# Autodesk Inventor assembly: DragBarLinkage3 Full Assembly
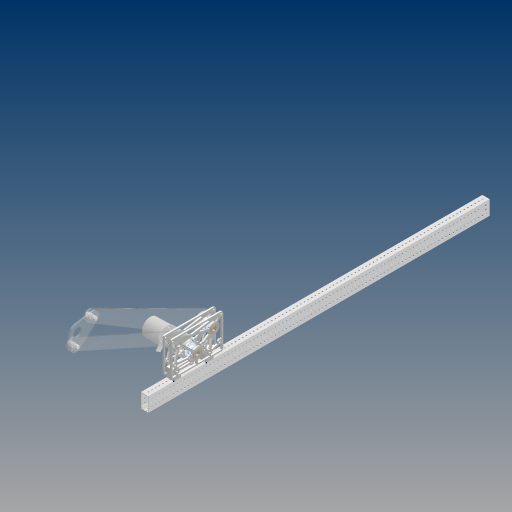
[picture p0: Inventor's stored thumbnail of the model, 512x512]
Saved by Autodesk Inventor 2024.3 (Build 283343000, 343)
## iProperties
Created: 2024-07-08
Part Number: DragBarLinkage3 Full Assembly
Document SubType Name: Assembly
Designer: Kenji
Author: Kenji
## Documents named in this file (21)
- C:\Users\Kenji\Documents\FRC\Offseason 2024\DragBarLinkage3\DragBarLinkage3 Full Assembly.iam
- C:\Users\Kenji\Documents\FRC\Offseason 2024\DragBarLinkage3\MAXPlanetary 3-Stage2.iam
- C:\Users\Kenji\Documents\FRC\Offseason 2024\DragBarLinkage3\DragBarLinkage3 Bar1.ipt
- C:\Users\Kenji\Documents\FRC\Offseason 2024\DragBarLinkage3\DragBarLinkage3 Bar2.ipt
- C:\Users\Kenji\Documents\FRC\Offseason 2024\DragBarLinkage3\DragBarLinkage3 Bar3.ipt
- C:\Users\Kenji\Documents\FRC\Offseason 2024\DragBarLinkage3\REV-21-2289.ipt
- C:\Users\Kenji\Documents\FRC\Offseason 2024\DragBarLinkage3\6655K14_Thrust Ball Bearing.ipt
- C:\Users\Kenji\Documents\FRC\Offseason 2024\DragBarLinkage3\57155K306_Stainless Steel Ball Bearing.ipt
- C:\Users\Kenji\Documents\FRC\Offseason 2024\DragBarLinkage3\91259A581_Alloy Steel Shoulder Screw.ipt
- C:\Users\Kenji\Documents\FRC\Offseason 2024\DragBarLinkage3\92141A226_18-8 Stainless Steel Washer.ipt
- C:\Users\Kenji\Documents\FRC\Offseason 2024\DragBarLinkage3\97135A414_High-Strength Steel Nylon-Insert Locknut.ipt
- C:\Users\Kenji\Documents\FRC\Offseason 2024\DragBarLinkage3\DragBarLinkage3 Bracket1.ipt
- C:\Users\Kenji\Documents\FRC\Offseason 2024\DragBarLinkage3\DragBarLinkage3 Billet.ipt
- C:\Users\Kenji\Documents\FRC\Offseason 2024\DragBarLinkage3\WCP-0754.ipt
- C:\Users\Kenji\Documents\FRC\Offseason 2024\DragBarLinkage3\WCP-0783 (1).ipt
- C:\Users\Kenji\Documents\FRC\Offseason 2024\DragBarLinkage3\1_2” Hex Bore Aluminum VersaHub (217-2592).ipt
- C:\Users\Kenji\Documents\FRC\Offseason 2024\DragBarLinkage3\5909K978_1-16 Thick Washe.ipt
- C:\Users\Kenji\Documents\FRC\Offseason 2024\DragBarLinkage3\5909K24_Needle-Roller Thrust Bearing.ipt
- C:\Users\Kenji\Documents\FRC\Offseason 2024\DragBarLinkage3\5909K951_Needle-Roller Thrust Bearing.ipt
- C:\Users\Kenji\Documents\FRC\Offseason 2024\DragBarLinkage3\5909K979_1-16 Thick Washe.ipt
- C:\Users\Kenji\Documents\FRC\Offseason 2024\DragBarLinkage3\5909K971_1-32 Thick Washe.ipt
## Components (36 placed, 20 different names)
1. MAXPlanetary 3-Stage2:1 [sub-assembly] — Mate:51, Mate:53, Mate:67
2. DragBarLinkage3 Bar1:1 — Mate:4, Mate:5, Mate:13, Mate:54, Mate:77, Mate:78, Mate:79
3. DragBarLinkage3 Bar2:1 — Mate:16, Mate:17, Mate:18, Mate:19, Mate:20, Mate:21, Mate:22, Mate:23
4. DragBarLinkage3 Bar3:1 — Mate:6, Mate:7, Mate:14, Mate:15, Mate:55, Mate:81, Mate:90, Mate:91, Mate:92
5. REV-21-2289:1 — Mate:41, Mate:42, Mate:43, Mate:44, Flush:1
6. 6655K14_Thrust Ball Bearing:1 — Mate:14, Mate:15, Mate:22, Mate:23
7. 6655K14_Thrust Ball Bearing:2 — Mate:12, Mate:13, Mate:20, Mate:21
8. 57155K306_Stainless Steel Ball Bearing:5 — Mate:16, Mate:18, Mate:36
9. 57155K306_Stainless Steel Ball Bearing:6 — Mate:6, Mate:7, Mate:26, Mate:27
10. 57155K306_Stainless Steel Ball Bearing:7 — Mate:4, Mate:5, Mate:12, Mate:24, Mate:25
11. 57155K306_Stainless Steel Ball Bearing:8 — Mate:17, Mate:19, Mate:31
12. 91259A581_Alloy Steel Shoulder Screw:1 — Mate:28, Mate:29, Mate:30
13. 91259A581_Alloy Steel Shoulder Screw:2 — Mate:32, Mate:33, Mate:34, Mate:35
14. 92141A226_18-8 Stainless Steel Washer:1 — Mate:24, Mate:25, Mate:28, Mate:29
15. 92141A226_18-8 Stainless Steel Washer:2 — Mate:26, Mate:27, Mate:32, Mate:33
16. 97135A414_High-Strength Steel Nylon-Insert Locknut:1 — Mate:30, Mate:31
17. 97135A414_High-Strength Steel Nylon-Insert Locknut:2 — Mate:34, Mate:35, Mate:36
18. DragBarLinkage3 Bracket1:2 — Mate:59, Mate:60, Mate:61, Mate:69, Mate:70, Mate:73, Mate:74
19. DragBarLinkage3 Billet:1 — Mate:42, Mate:44, Flush:2, Mate:50, Mate:58, Mate:60, Mate:61
20. DragBarLinkage3 Billet:2 — Mate:41, Mate:43, Flush:1, Flush:2, Mate:57, Mate:59
21. DragBarLinkage3 Bracket1:3 — Mate:50, Mate:51, Mate:53, Mate:54, Mate:55, Mate:57, Mate:58, Mate:66, Mate:67, Mate:68, Mate:71, Mate:72, Mate:76, Mate:80, Mate:82, Mate:83
22. 57155K306_Stainless Steel Ball Bearing:9 — Mate:81, Mate:82, Mate:88, Mate:89
23. 57155K306_Stainless Steel Ball Bearing:10 — Mate:80, Mate:83
24. WCP-0754:1 — Mate:66, Mate:76
25. WCP-0754:2 — Mate:68, Mate:75
26. WCP-0783 (1):1 — Mate:73, Mate:74
27. WCP-0783 (1):2 — Mate:71, Mate:72, Mate:75, Mate:98, Mate:99
28. WCP-0783 (1):4 — Mate:69, Mate:70
29. 1_2” Hex Bore Aluminum VersaHub (217-2592):1 — Mate:77, Mate:78, Mate:79
30. 5909K978_1-16 Thick Washe:1 — Mate:84, Mate:87, Mate:88, Mate:90
31. 5909K978_1-16 Thick Washe:2 — Mate:85, Mate:86, Mate:89
32. 5909K24_Needle-Roller Thrust Bearing:1 — Mate:84, Mate:85, Mate:86, Mate:87
33. 57155K306_Stainless Steel Ball Bearing:11 — Mate:91, Mate:92
34. 5909K951_Needle-Roller Thrust Bearing:1 — Mate:93, Mate:95, Mate:96, Mate:97
35. 5909K979_1-16 Thick Washe:1 — Mate:93, Mate:95
36. 5909K971_1-32 Thick Washe:1 — Mate:96, Mate:97, Mate:98, Mate:99
## Relationships (78: Mate 76, Flush 2)
- Mate:4: DragBarLinkage3 Bar1:1 ↔ 57155K306_Stainless Steel Ball Bearing:7
- Mate:5: DragBarLinkage3 Bar1:1 ↔ 57155K306_Stainless Steel Ball Bearing:7
- Mate:6: DragBarLinkage3 Bar3:1 ↔ 57155K306_Stainless Steel Ball Bearing:6
- Mate:7: DragBarLinkage3 Bar3:1 ↔ 57155K306_Stainless Steel Ball Bearing:6
- Mate:12: 6655K14_Thrust Ball Bearing:2 ↔ 57155K306_Stainless Steel Ball Bearing:7
- Mate:13: DragBarLinkage3 Bar1:1 ↔ 6655K14_Thrust Ball Bearing:2
- Mate:14: DragBarLinkage3 Bar3:1 ↔ 6655K14_Thrust Ball Bearing:1
- Mate:15: DragBarLinkage3 Bar3:1 ↔ 6655K14_Thrust Ball Bearing:1
- Mate:16: DragBarLinkage3 Bar2:1 ↔ 57155K306_Stainless Steel Ball Bearing:5
- Mate:17: DragBarLinkage3 Bar2:1 ↔ 57155K306_Stainless Steel Ball Bearing:8
- Mate:18: DragBarLinkage3 Bar2:1 ↔ 57155K306_Stainless Steel Ball Bearing:5
- Mate:19: DragBarLinkage3 Bar2:1 ↔ 57155K306_Stainless Steel Ball Bearing:8
- Mate:20: DragBarLinkage3 Bar2:1 ↔ 6655K14_Thrust Ball Bearing:2
- Mate:21: DragBarLinkage3 Bar2:1 ↔ 6655K14_Thrust Ball Bearing:2
- Mate:22: DragBarLinkage3 Bar2:1 ↔ 6655K14_Thrust Ball Bearing:1
- Mate:23: DragBarLinkage3 Bar2:1 ↔ 6655K14_Thrust Ball Bearing:1
- Mate:24: 57155K306_Stainless Steel Ball Bearing:7 ↔ 92141A226_18-8 Stainless Steel Washer:1
- Mate:25: 57155K306_Stainless Steel Ball Bearing:7 ↔ 92141A226_18-8 Stainless Steel Washer:1
- Mate:26: 57155K306_Stainless Steel Ball Bearing:6 ↔ 92141A226_18-8 Stainless Steel Washer:2
- Mate:27: 57155K306_Stainless Steel Ball Bearing:6 ↔ 92141A226_18-8 Stainless Steel Washer:2
- Mate:28: 91259A581_Alloy Steel Shoulder Screw:1 ↔ 92141A226_18-8 Stainless Steel Washer:1
- Mate:29: 91259A581_Alloy Steel Shoulder Screw:1 ↔ 92141A226_18-8 Stainless Steel Washer:1
- Mate:30: 91259A581_Alloy Steel Shoulder Screw:1 ↔ 97135A414_High-Strength Steel Nylon-Insert Locknut:1
- Mate:31: 57155K306_Stainless Steel Ball Bearing:8 ↔ 97135A414_High-Strength Steel Nylon-Insert Locknut:1
- Mate:32: 91259A581_Alloy Steel Shoulder Screw:2 ↔ 92141A226_18-8 Stainless Steel Washer:2
- Mate:33: 91259A581_Alloy Steel Shoulder Screw:2 ↔ 92141A226_18-8 Stainless Steel Washer:2
- Mate:34: 91259A581_Alloy Steel Shoulder Screw:2 ↔ 97135A414_High-Strength Steel Nylon-Insert Locknut:2
- Mate:35: 91259A581_Alloy Steel Shoulder Screw:2 ↔ 97135A414_High-Strength Steel Nylon-Insert Locknut:2
- Mate:36: 57155K306_Stainless Steel Ball Bearing:5 ↔ 97135A414_High-Strength Steel Nylon-Insert Locknut:2
- Mate:41: REV-21-2289:1 ↔ DragBarLinkage3 Billet:2
- Mate:42: REV-21-2289:1 ↔ DragBarLinkage3 Billet:1
- Mate:43: REV-21-2289:1 ↔ DragBarLinkage3 Billet:2
- Mate:44: REV-21-2289:1 ↔ DragBarLinkage3 Billet:1
- Flush:1: REV-21-2289:1 ↔ DragBarLinkage3 Billet:2
- Flush:2: DragBarLinkage3 Billet:1 ↔ DragBarLinkage3 Billet:2
- Mate:50: DragBarLinkage3 Billet:1 ↔ DragBarLinkage3 Bracket1:3
- Mate:51: MAXPlanetary 3-Stage2:1 ↔ DragBarLinkage3 Bracket1:3
- Mate:53: MAXPlanetary 3-Stage2:1 ↔ DragBarLinkage3 Bracket1:3
- Mate:54: DragBarLinkage3 Bar1:1 ↔ DragBarLinkage3 Bracket1:3
- Mate:55: DragBarLinkage3 Bar3:1 ↔ DragBarLinkage3 Bracket1:3
- Mate:57: DragBarLinkage3 Billet:2 ↔ DragBarLinkage3 Bracket1:3
- Mate:58: DragBarLinkage3 Billet:1 ↔ DragBarLinkage3 Bracket1:3
- Mate:59: DragBarLinkage3 Bracket1:2 ↔ DragBarLinkage3 Billet:2
- Mate:60: DragBarLinkage3 Bracket1:2 ↔ DragBarLinkage3 Billet:1
- Mate:61: DragBarLinkage3 Bracket1:2 ↔ DragBarLinkage3 Billet:1
- Mate:66: DragBarLinkage3 Bracket1:3 ↔ WCP-0754:1
- Mate:67: MAXPlanetary 3-Stage2:1 ↔ DragBarLinkage3 Bracket1:3
- Mate:68: DragBarLinkage3 Bracket1:3 ↔ WCP-0754:2
- Mate:69: DragBarLinkage3 Bracket1:2 ↔ WCP-0783 (1):4
- Mate:70: DragBarLinkage3 Bracket1:2 ↔ WCP-0783 (1):4
- Mate:71: DragBarLinkage3 Bracket1:3 ↔ WCP-0783 (1):2
- Mate:72: DragBarLinkage3 Bracket1:3 ↔ WCP-0783 (1):2
- Mate:73: DragBarLinkage3 Bracket1:2 ↔ WCP-0783 (1):1
- Mate:74: DragBarLinkage3 Bracket1:2 ↔ WCP-0783 (1):1
- Mate:75: WCP-0754:2 ↔ WCP-0783 (1):2
- Mate:76: DragBarLinkage3 Bracket1:3 ↔ WCP-0754:1
- Mate:77: DragBarLinkage3 Bar1:1 ↔ 1_2” Hex Bore Aluminum VersaHub (217-2592):1
- Mate:78: DragBarLinkage3 Bar1:1 ↔ 1_2” Hex Bore Aluminum VersaHub (217-2592):1
- Mate:79: DragBarLinkage3 Bar1:1 ↔ 1_2” Hex Bore Aluminum VersaHub (217-2592):1
- Mate:80: DragBarLinkage3 Bracket1:3 ↔ 57155K306_Stainless Steel Ball Bearing:10
- Mate:81: DragBarLinkage3 Bar3:1 ↔ 57155K306_Stainless Steel Ball Bearing:9
- Mate:82: DragBarLinkage3 Bracket1:3 ↔ 57155K306_Stainless Steel Ball Bearing:9
- Mate:83: DragBarLinkage3 Bracket1:3 ↔ 57155K306_Stainless Steel Ball Bearing:10
- Mate:84: 5909K978_1-16 Thick Washe:1 ↔ 5909K24_Needle-Roller Thrust Bearing:1
- Mate:85: 5909K978_1-16 Thick Washe:2 ↔ 5909K24_Needle-Roller Thrust Bearing:1
- Mate:86 (0.4953 mm): 5909K978_1-16 Thick Washe:2 ↔ 5909K24_Needle-Roller Thrust Bearing:1
- Mate:87 (0.4953 mm): 5909K978_1-16 Thick Washe:1 ↔ 5909K24_Needle-Roller Thrust Bearing:1
- Mate:88: 57155K306_Stainless Steel Ball Bearing:9 ↔ 5909K978_1-16 Thick Washe:1
- Mate:89: 57155K306_Stainless Steel Ball Bearing:9 ↔ 5909K978_1-16 Thick Washe:2
- Mate:90: DragBarLinkage3 Bar3:1 ↔ 5909K978_1-16 Thick Washe:1
- Mate:91: DragBarLinkage3 Bar3:1 ↔ 57155K306_Stainless Steel Ball Bearing:11
- Mate:92: DragBarLinkage3 Bar3:1 ↔ 57155K306_Stainless Steel Ball Bearing:11
- Mate:93: 5909K951_Needle-Roller Thrust Bearing:1 ↔ 5909K979_1-16 Thick Washe:1
- Mate:95 (0.602 mm): 5909K951_Needle-Roller Thrust Bearing:1 ↔ 5909K979_1-16 Thick Washe:1
- Mate:96: 5909K951_Needle-Roller Thrust Bearing:1 ↔ 5909K971_1-32 Thick Washe:1
- Mate:97 (0.602 mm): 5909K951_Needle-Roller Thrust Bearing:1 ↔ 5909K971_1-32 Thick Washe:1
- Mate:98: WCP-0783 (1):2 ↔ 5909K971_1-32 Thick Washe:1
- Mate:99: WCP-0783 (1):2 ↔ 5909K971_1-32 Thick Washe:1
